# Autodesk Inventor assembly: WheelAssembly
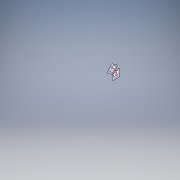
[picture p0: Inventor's stored thumbnail of the model, 180x180]
Saved by Autodesk Inventor 2016 (Build 200138000, 138)
## iProperties
Created: 2016-09-10
Part Number: WheelAssembly
Document SubType Name: Assembly
Designer: RoboticsUser
Author: RoboticsUser
## Documents named in this file (5)
- C:\Users\RoboticsUser\Desktop\2015-16 CAD\custom cad parts\WheelAssembly.iam
- C:\Robotics\CAD\2015-16\custom cad parts\am-2648_4inWheel8mmHub.ipt
- C:\Robotics\CAD\2015-16\COTSParts\Actobotics\545 parts\545556.ipt
- C:\Robotics\CAD\2015-16\COTSParts\Actobotics\615 parts\615102.ipt
- C:\Robotics\CAD\2015-16\COTSParts\Actobotics\634 parts\634080.ipt
## Components (7 placed, 4 different names)
1. 545556:5 — Insert:8, Insert:10
2. am-2648_4inWheel8mmHub:2 — Insert:2, Insert:10
3. 545556:2 — Insert:2, Insert:9
4. 634080:1
5. 615102:3
6. 615102:4 — Insert:8
7. 634080:2 — Insert:9
## Relationships (4: Insert 4)
- Insert:2 (3.175 mm): am-2648_4inWheel8mmHub:2 ↔ 545556:2
- Insert:8: 545556:5 ↔ 615102:4
- Insert:9 (-12.7 mm): 545556:2 ↔ 634080:2
- Insert:10 (3.175 mm): 545556:5 ↔ am-2648_4inWheel8mmHub:2
